# Autodesk Inventor assembly: 조립품1
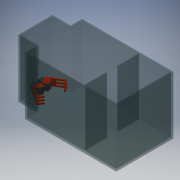
[picture p0: Inventor's stored thumbnail of the model, 180x180]
Saved by Autodesk Inventor 2019 (Build 230136000, 136)
## iProperties
Created: 2019-03-05
Part Number: 조립품1
Material: 일반
Document SubType Name: Assembly
Designer: Jeong Ji Hoon
Author: Jeong Ji Hoon
## Documents named in this file (4)
- D:\ChoiLab\과제\Lobsterbot_Space\조립품1.iam
- D:\ChoiLab\과제\Lobsterbot_Space\Space.ipt
- D:\ChoiLab\과제\Lobsterbot_Space\claw.ipt
- D:\ChoiLab\과제\Lobsterbot_Space\Motor.ipt
## Components (5 placed, 3 different names)
1. Space:1 — 강체:1, 강체:2
2. claw:1 — 회전:1
3. Motor:1 — 회전:1, 강체:1
4. claw:2
5. Motor:2 — 강체:2
## Relationships (4: RevoluteJoint 2, WeldJoint 2)
- 회전:1 [RevoluteJoint]: claw:1 ↔ Motor:1
- 강체:1 [WeldJoint]: Space:1 ↔ Motor:1
- [RevoluteJoint]: claw:2 ↔ Motor:2
- 강체:2 [WeldJoint]: Space:1 ↔ Motor:2
## Named parameters: d10_d0 = 0 mm, d11_d1 = 149 deg
